# Autodesk Inventor assembly: Structure
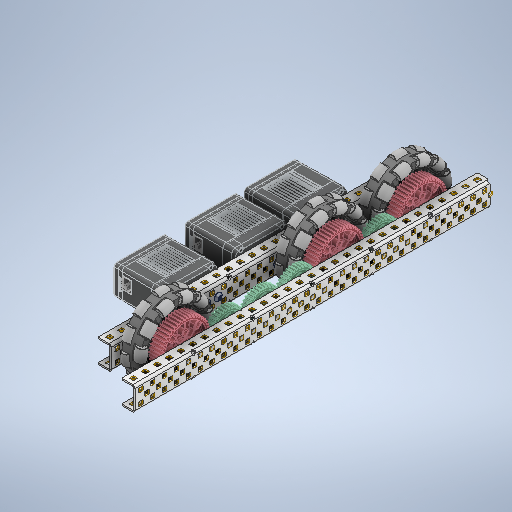
[picture p0: Inventor's stored thumbnail of the model, 512x512]
Saved by Autodesk Inventor 2025.2 (Build 292293000, 293)
## iProperties
Created: 2025-03-28
Part Number: Structure
Document SubType Name: Assembly
Designer: avere
Author: avere
## Documents named in this file (10)
- D:\vex\cad\v5\Drivetrain\Drivebay Left\!Drivebay Left.iam
- Drivebay.iam
- D:\vex\cad\VEX-CAD-Inventor\Structure\C Channel\Aluminum 1x2x1\Alu C 1x2x1x30.ipt
- D:\vex\cad\VEX-CAD-Inventor\Structure\C Channel\Aluminum 1x2x1\Alu C 1x2x1x26.ipt
- D:\vex\cad\VEX-CAD-Inventor\Structure\C Channel\Aluminum 1x2x1\Alu C 1x2x1x5.ipt
- D:\vex\cad\VEX-CAD-Inventor\Motion\Shaft LS\Bearing Flat Low Profile.ipt
- D:\vex\cad\VEX-CAD-Inventor\Electronics\Motors with Screws.iam
- D:\vex\cad\VEX-CAD-Inventor\Electronics\Motors with Screws\SteelM-StarS.iam
- D:\vex\cad\v5\Drivetrain\Drivebay Left\Wheel Hub.iam
- D:\vex\cad\v5\Drivetrain\Drivebay Left\Gear Hub.iam
## Components (21 placed, 7 different names)
1. Alu C 1x2x1x30:1 — Flush:1, Mate:1, Insert:2, Mate:3, Mate:7, Mate:8, Insert:6, Mate:9, Insert:7, Mate:10, Insert:9, Mate:11, Insert:10, Mate:12, Mate:13, Mate:14, Insert:12, Mate:15
2. Alu C 1x2x1x26:1 — Flush:1, Mate:1, Insert:1, Mate:2, Insert:13, Mate:16, Insert:14, Mate:17, Insert:15, Mate:18
3. Alu C 1x2x1x5:1 — Insert:1, Mate:2, Insert:2, Mate:3
4. Bearing Flat Low Profile:1 — Insert:6, Mate:9
5. SteelM-StarS:1 [sub-assembly] — Insert:13, Mate:16
6. Wheel Hub:1 [sub-assembly] — Mate:7, Mate:8
7. Bearing Flat Low Profile:9 — Insert:10, Mate:12
8. Bearing Flat Low Profile:11 — Insert:12, Mate:15
9. Gear Hub:4 [sub-assembly]
10. SteelM-StarS:2 [sub-assembly] — Insert:14, Mate:17
11. SteelM-StarS:3 [sub-assembly] — Insert:15, Mate:18
12. Gear Hub:1 [sub-assembly] — Insert:8
13. Bearing Flat Low Profile:5 — Insert:7, Mate:10, Insert:8
14. Gear Hub:2 [sub-assembly]
15. Bearing Flat Low Profile:6
16. Gear Hub:3 [sub-assembly]
17. Bearing Flat Low Profile:7
18. Bearing Flat Low Profile:8 — Insert:9, Mate:11
19. Wheel Hub:2 [sub-assembly] — Mate:13, Mate:14
20. Bearing Flat Low Profile:10
21. Wheel Hub:3 [sub-assembly]
## Component patterns: (3 elements, first: Gear Hub:1 + Bearing Flat Low Profile:5), (2 elements, first: Bearing Flat Low Profile:8 + Wheel Hub:2)
## Relationships (28: Mate 15, Insert 12, Flush 1)
- Flush:1: Alu C 1x2x1x30:1 ↔ Alu C 1x2x1x26:1
- Mate:1: Alu C 1x2x1x30:1 ↔ Alu C 1x2x1x26:1
- Insert:1: Alu C 1x2x1x26:1 ↔ Alu C 1x2x1x5:1
- Mate:2: Alu C 1x2x1x26:1 ↔ Alu C 1x2x1x5:1
- Insert:2: Alu C 1x2x1x30:1 ↔ Alu C 1x2x1x5:1
- Mate:3: Alu C 1x2x1x30:1 ↔ Alu C 1x2x1x5:1
- Mate:7 (1.5875 mm): Alu C 1x2x1x30:1 ↔ Wheel Hub:1
- Mate:8: Alu C 1x2x1x30:1 ↔ Wheel Hub:1
- Insert:6: Alu C 1x2x1x30:1 ↔ Bearing Flat Low Profile:1
- Mate:9: Alu C 1x2x1x30:1 ↔ Bearing Flat Low Profile:1
- Insert:7: Alu C 1x2x1x30:1 ↔ Bearing Flat Low Profile:5
- Mate:10: Alu C 1x2x1x30:1 ↔ Bearing Flat Low Profile:5
- Insert:8 (7.1437 mm): Gear Hub:1 ↔ Bearing Flat Low Profile:5
- Insert:9: Alu C 1x2x1x30:1 ↔ Bearing Flat Low Profile:8
- Mate:11: Alu C 1x2x1x30:1 ↔ Bearing Flat Low Profile:8
- Insert:10: Alu C 1x2x1x30:1 ↔ Bearing Flat Low Profile:9
- Mate:12: Alu C 1x2x1x30:1 ↔ Bearing Flat Low Profile:9
- Mate:13 (1.5875 mm): Alu C 1x2x1x30:1 ↔ Wheel Hub:2
- Mate:14: Alu C 1x2x1x30:1 ↔ Wheel Hub:2
- [Insert] (7.1437 mm): Bearing Flat Low Profile:11 ↔ Gear Hub:4
- Insert:12: Alu C 1x2x1x30:1 ↔ Bearing Flat Low Profile:11
- Mate:15: Alu C 1x2x1x30:1 ↔ Bearing Flat Low Profile:11
- Insert:13: Alu C 1x2x1x26:1 ↔ SteelM-StarS:1
- Mate:16: Alu C 1x2x1x26:1 ↔ SteelM-StarS:1
- Insert:14: Alu C 1x2x1x26:1 ↔ SteelM-StarS:2
- Mate:17: Alu C 1x2x1x26:1 ↔ SteelM-StarS:2
- Insert:15: Alu C 1x2x1x26:1 ↔ SteelM-StarS:3
- Mate:18: Alu C 1x2x1x26:1 ↔ SteelM-StarS:3
## Named parameters: d74_d59 = 7.14375 mm
